# Autodesk Inventor assembly: Slider_crank_mechanism
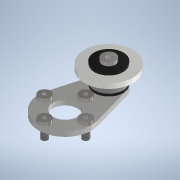
[picture p0: Inventor's stored thumbnail of the model, 180x180]
Saved by Autodesk Inventor 2020 (Build 240168000, 168)
## iProperties
Created: 2021-09-06
Part Number: Slider_crank_mechanism
Document SubType Name: Assembly
Designer: Masato Kubotera
Mass: 2.53036 g
Surface Area: 18.5815 cm^2
Volume: 1.13409 cm^3
Density: 2.23118 g/cm^3
Author: Masato Kubotera
## Documents named in this file (10)
- C:\Users\Masato\Documents\Inventor\CIT Brains_Inventor\OpenPlatform_ver3_0\LowerBody\Slider_crank\Slider_crank_mechanism.iam
- C:\Users\Masato\Documents\Inventor\CIT Brains_Inventor\OpenPlatform_ver3_0\LowerBody\Slider_crank\Slider_crank_horn.ipt
- C:\Users\Masato\Documents\Inventor\CIT Brains_Inventor\OpenPlatform_ver3_0\Ready_Made\UUW-0312-10BH.ipt
- C:\Users\Masato\Documents\Inventor\CIT Brains_Inventor\OpenPlatform_ver3_0\Ready_Made\SF319.ipt
- C:\Users\Masato\Documents\Inventor\CIT Brains_Inventor\OpenPlatform_ver3_0\Ready_Made\LED-0606.ipt
- C:\Users\Masato\Documents\Inventor\CIT Brains_Inventor\OpenPlatform_ver3_0\Ready_Made\Screw\M2_6-6.ipt
- C:\Users\Masato\Documents\Inventor\CIT Brains_Inventor\OpenPlatform_ver3_0\Ready_Made\Screw\M3-10.ipt
- C:\Users\Masato\Documents\Inventor\CIT Brains_Inventor\OpenPlatform_ver3_0\Ready_Made\TT-1020-20.ipt
- C:\Users\Masato\Documents\Inventor\CIT Brains_Inventor\OpenPlatform_ver3_0\Ready_Made\ARU-306_5SMO.ipt
- ARU-306S.ipt
## Components (12 placed, 8 different names)
1. Slider_crank_horn:1 — 挿入:1, 挿入:9, 挿入:13, 挿入:14, 挿入:15, 挿入:16
2. UUW-0312-10BH:1 — 挿入:1, 挿入:17, 挿入:22
3. UUW-0312-10BH:2 — 挿入:20, 挿入:21, 挿入:23
4. SF319:1 — 挿入:9
5. LED-0606:1 — 挿入:17
6. M2_6-6:1 — 挿入:13
7. M2_6-6:2 — 挿入:14
8. M2_6-6:3 — 挿入:15
9. M2_6-6:4 — 挿入:16
10. M3-10:1 — 挿入:20
11. TT-1020-20:1 — 挿入:21
12. ARU-306S:1 — 挿入:22, 挿入:23
## Relationships (11: Insert 11)
- 挿入:1 [Insert]: Slider_crank_horn:1 ↔ UUW-0312-10BH:1
- 挿入:9 [Insert]: Slider_crank_horn:1 ↔ SF319:1
- 挿入:13 [Insert]: Slider_crank_horn:1 ↔ M2_6-6:1
- 挿入:14 [Insert]: Slider_crank_horn:1 ↔ M2_6-6:2
- 挿入:15 [Insert]: Slider_crank_horn:1 ↔ M2_6-6:3
- 挿入:16 [Insert]: Slider_crank_horn:1 ↔ M2_6-6:4
- 挿入:17 [Insert]: UUW-0312-10BH:1 ↔ LED-0606:1
- 挿入:20 [Insert]: UUW-0312-10BH:2 ↔ M3-10:1
- 挿入:21 [Insert]: UUW-0312-10BH:2 ↔ TT-1020-20:1
- 挿入:22 [Insert]: UUW-0312-10BH:1 ↔ ARU-306S:1
- 挿入:23 [Insert]: UUW-0312-10BH:2 ↔ ARU-306S:1
